# Autodesk Inventor assembly: Track Frame Assembly
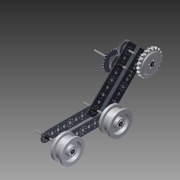
[picture p0: Inventor's stored thumbnail of the model, 180x180]
Saved by Autodesk Inventor 2015 (Build 190159000, 159)
## iProperties
Created: 2015-09-27
Part Number: Track Frame Assembly
Document SubType Name: Assembly
Designer: Jing-Chen
Author: Jing-Chen
## Documents named in this file (14)
- C:\Users\Jing-Chen\Desktop\Bionic Hybrids 2016\Bionic-Hybrids\CAD\Drivetrain\Sub-Assemblies\Track Frame Assembly.iam
- C:\Users\Jing-Chen\Desktop\Bionic Hybrids 2016\Bionic-Hybrids\Stock\Bracket-U9 - 739067.ipt
- C:\Users\Jing-Chen\Desktop\Bionic Hybrids 2016\Bionic-Hybrids\CAD\Drivetrain\Sub-Assemblies\Track Idler Assembly.iam
- C:\Users\Jing-Chen\Desktop\Bionic Hybrids 2016\Bionic-Hybrids\Stock\Axle-100mm - 739088.ipt
- C:\Users\Jing-Chen\Desktop\Bionic Hybrids 2016\Bionic-Hybrids\Stock\Bearing-Thrust - 739091.ipt
- C:\Users\Jing-Chen\Desktop\Bionic Hybrids 2016\Bionic-Hybrids\Stock\Shaft Collar-Setscrew, Axle - 739092.iam
- C:\Users\Jing-Chen\Desktop\Bionic Hybrids 2016\Bionic-Hybrids\Stock\Track Sprocket - 736468.ipt
- C:\Users\Jing-Chen\Desktop\Bionic Hybrids 2016\Bionic-Hybrids\Stock\Shaft Collar-Setscrew, Axle, Mountable - 739172.iam
- C:\Users\Jing-Chen\Desktop\Bionic Hybrids 2016\Bionic-Hybrids\Stock\Plate-9x1 - 739272.ipt
- C:\Users\Jing-Chen\Desktop\Bionic Hybrids 2016\Bionic-Hybrids\Stock\Spacer 3.125mm- 739100.ipt
- C:\Users\Jing-Chen\Desktop\Bionic Hybrids 2016\Bionic-Hybrids\Stock\Gear-40 tooth - 731901.ipt
- C:\Users\Jing-Chen\Desktop\Bionic Hybrids 2016\Bionic-Hybrids\Stock\Plate-1x1 - 739387.ipt
- C:\Users\Jing-Chen\Desktop\Bionic Hybrids 2016\Bionic-Hybrids\Stock\Chain Sprocket-24 tooth - 739169.ipt
- C:\Users\Jing-Chen\Desktop\Bionic Hybrids 2016\Bionic-Hybrids\Stock\Screw 0.5in - 739097.ipt
## Components (36 placed, 13 different names)
1. Bracket-U9 - 739067:1 — Mate:16, Mate:17, Mate:18, Mate:19, Mate:20, Mate:21, Mate:44, Mate:46, Mate:60, Mate:61, Mate:63, Flush:6, Mate:66, Mate:67, Mate:88, Mate:89, Mate:90, Mate:91, Mate:93, Mate:94, Mate:95
2. Track Idler Assembly:1 [sub-assembly] — Mate:2, Flush:1, Mate:43
3. Axle-100mm - 739088:1 — Mate:2, Flush:1, Mate:11, Mate:41
4. Shaft Collar-Setscrew, Axle - 739092:1 [sub-assembly] — Mate:11, Mate:42
5. Track Sprocket - 736468:1 — Mate:13, Mate:15, Mate:23, Mate:24, Mate:105
6. Shaft Collar-Setscrew, Axle, Mountable - 739172:1 [sub-assembly] — Mate:13, Mate:15, Mate:22, Mate:105, Mate:106, Angle:3
7. Plate-9x1 - 739272:1 — Mate:16, Mate:19, Mate:21, Mate:37, Mate:38, Mate:45, Flush:4, Flush:5, Mate:53
8. Plate-9x1 - 739272:2 — Mate:17, Mate:18, Mate:20, Mate:39, Mate:40, Mate:47
9. Axle-100mm - 739088:2 — Mate:22, Flush:2, Mate:58, Mate:92, Mate:99, Mate:100, Mate:101, Angle:2, Angle:3
10. Bearing-Thrust - 739091:4 — Mate:23, Mate:24, Flush:2
11. Bearing-Thrust - 739091:5 — Mate:44, Mate:45, Mate:48, Mate:50
12. Bearing-Thrust - 739091:6 — Mate:39, Mate:40, Mate:41, Mate:42
13. Bearing-Thrust - 739091:10 — Mate:46, Mate:47, Mate:52
14. Bearing-Thrust - 739091:11 — Mate:37, Mate:38, Mate:43
15. Axle-100mm - 739088:3 — Mate:48, Mate:49, Flush:3, Mate:51
16. Track Idler Assembly:2 [sub-assembly] — Mate:49, Mate:50, Flush:3
17. Shaft Collar-Setscrew, Axle - 739092:2 [sub-assembly] — Mate:51, Mate:52
18. Gear-40 tooth - 731901:1 — Mate:55, Mate:57, Mate:64, Rotation:1, Mate:84, Mate:85, Mate:86, Mate:87
19. Gear-40 tooth - 731901:2 — Mate:73, Mate:74, Mate:75, Mate:76, Rotation:1
20. Shaft Collar-Setscrew, Axle, Mountable - 739172:2 [sub-assembly] — Mate:55, Mate:57, Mate:58, Mate:63, Mate:64, Angle:2
21. Shaft Collar-Setscrew, Axle, Mountable - 739172:4 [sub-assembly] — Mate:60, Mate:61, Mate:65, Mate:66, Angle:1
22. Axle-100mm - 739088:4 — Mate:65, Flush:6, Mate:68, Mate:69, Mate:71, Mate:77, Mate:78, Angle:1, Mate:82
23. Plate-1x1 - 739387:1 — Mate:67, Mate:68, Mate:70
24. Bearing-Thrust - 739091:12 — Mate:69, Mate:70, Mate:72
25. Spacer 3.125mm- 739100:3 — Mate:71, Mate:72, Mate:76
26. Shaft Collar-Setscrew, Axle, Mountable - 739172:6 [sub-assembly] — Mate:73, Mate:74, Mate:75, Mate:77, Mate:79, Mate:80, Mate:81
27. Chain Sprocket-24 tooth - 739169:1 — Mate:78, Mate:79, Mate:80, Mate:81, Mate:83
28. Spacer 3.125mm- 739100:4 — Mate:82, Mate:83
29. Screw 0.5in - 739097:1 — Mate:84, Mate:86
30. Screw 0.5in - 739097:2 — Mate:85, Mate:87
31. Screw 0.5in - 739097:3 — Mate:88, Mate:90
32. Screw 0.5in - 739097:4 — Mate:89, Mate:91
33. Shaft Collar-Setscrew, Axle, Mountable - 739172:7 [sub-assembly] — Mate:92, Mate:93, Mate:94, Mate:95, Mate:104
34. Spacer 3.125mm- 739100:5 — Mate:101, Mate:102, Mate:104
35. Spacer 3.125mm- 739100:6 — Mate:100, Mate:102, Mate:103
36. Spacer 3.125mm- 739100:7 — Mate:99, Mate:103, Mate:106
## Relationships (86: Mate 76, Flush 6, Angle 3, RelateRotation 1)
- Mate:2: Track Idler Assembly:1 ↔ Axle-100mm - 739088:1
- Flush:1: Track Idler Assembly:1 ↔ Axle-100mm - 739088:1
- Mate:11: Axle-100mm - 739088:1 ↔ Shaft Collar-Setscrew, Axle - 739092:1
- Mate:13: Track Sprocket - 736468:1 ↔ Shaft Collar-Setscrew, Axle, Mountable - 739172:1
- Mate:15: Track Sprocket - 736468:1 ↔ Shaft Collar-Setscrew, Axle, Mountable - 739172:1
- Mate:16: Bracket-U9 - 739067:1 ↔ Plate-9x1 - 739272:1
- Mate:17: Bracket-U9 - 739067:1 ↔ Plate-9x1 - 739272:2
- Mate:18: Bracket-U9 - 739067:1 ↔ Plate-9x1 - 739272:2
- Mate:19: Bracket-U9 - 739067:1 ↔ Plate-9x1 - 739272:1
- Mate:20: Bracket-U9 - 739067:1 ↔ Plate-9x1 - 739272:2
- Mate:21: Bracket-U9 - 739067:1 ↔ Plate-9x1 - 739272:1
- Mate:22: Shaft Collar-Setscrew, Axle, Mountable - 739172:1 ↔ Axle-100mm - 739088:2
- Mate:23: Track Sprocket - 736468:1 ↔ Bearing-Thrust - 739091:4
- Mate:24: Track Sprocket - 736468:1 ↔ Bearing-Thrust - 739091:4
- Flush:2: Axle-100mm - 739088:2 ↔ Bearing-Thrust - 739091:4
- Mate:37: Plate-9x1 - 739272:1 ↔ Bearing-Thrust - 739091:11
- Mate:38: Plate-9x1 - 739272:1 ↔ Bearing-Thrust - 739091:11
- Mate:39: Plate-9x1 - 739272:2 ↔ Bearing-Thrust - 739091:6
- Mate:40: Plate-9x1 - 739272:2 ↔ Bearing-Thrust - 739091:6
- Mate:41: Axle-100mm - 739088:1 ↔ Bearing-Thrust - 739091:6
- Mate:42: Shaft Collar-Setscrew, Axle - 739092:1 ↔ Bearing-Thrust - 739091:6
- Mate:43: Track Idler Assembly:1 ↔ Bearing-Thrust - 739091:11
- Mate:44: Bracket-U9 - 739067:1 ↔ Bearing-Thrust - 739091:5
- Mate:45: Plate-9x1 - 739272:1 ↔ Bearing-Thrust - 739091:5
- Mate:46: Bracket-U9 - 739067:1 ↔ Bearing-Thrust - 739091:10
- Mate:47: Plate-9x1 - 739272:2 ↔ Bearing-Thrust - 739091:10
- Mate:48: Bearing-Thrust - 739091:5 ↔ Axle-100mm - 739088:3
- Mate:49: Axle-100mm - 739088:3 ↔ Track Idler Assembly:2
- Mate:50: Bearing-Thrust - 739091:5 ↔ Track Idler Assembly:2
- Flush:3: Axle-100mm - 739088:3 ↔ Track Idler Assembly:2
- Mate:51: Axle-100mm - 739088:3 ↔ Shaft Collar-Setscrew, Axle - 739092:2
- Mate:52: Bearing-Thrust - 739091:10 ↔ Shaft Collar-Setscrew, Axle - 739092:2
- Flush:4: Plate-9x1 - 739272:1
- Flush:5: Plate-9x1 - 739272:1
- Mate:53: Plate-9x1 - 739272:1
- Mate:55: Gear-40 tooth - 731901:1 ↔ Shaft Collar-Setscrew, Axle, Mountable - 739172:2
- Mate:57: Gear-40 tooth - 731901:1 ↔ Shaft Collar-Setscrew, Axle, Mountable - 739172:2
- Mate:58: Axle-100mm - 739088:2 ↔ Shaft Collar-Setscrew, Axle, Mountable - 739172:2
- Mate:60: Bracket-U9 - 739067:1 ↔ Shaft Collar-Setscrew, Axle, Mountable - 739172:4
- Mate:61: Bracket-U9 - 739067:1 ↔ Shaft Collar-Setscrew, Axle, Mountable - 739172:4
- Mate:63: Bracket-U9 - 739067:1 ↔ Shaft Collar-Setscrew, Axle, Mountable - 739172:2
- Mate:64: Gear-40 tooth - 731901:1 ↔ Shaft Collar-Setscrew, Axle, Mountable - 739172:2
- Mate:65: Shaft Collar-Setscrew, Axle, Mountable - 739172:4 ↔ Axle-100mm - 739088:4
- Flush:6: Bracket-U9 - 739067:1 ↔ Axle-100mm - 739088:4
- Mate:66: Bracket-U9 - 739067:1 ↔ Shaft Collar-Setscrew, Axle, Mountable - 739172:4
- Mate:67: Bracket-U9 - 739067:1 ↔ Plate-1x1 - 739387:1
- Mate:68: Axle-100mm - 739088:4 ↔ Plate-1x1 - 739387:1
- Mate:69: Axle-100mm - 739088:4 ↔ Bearing-Thrust - 739091:12
- Mate:70: Plate-1x1 - 739387:1 ↔ Bearing-Thrust - 739091:12
- Mate:71: Axle-100mm - 739088:4 ↔ Spacer 3.125mm- 739100:3
- Mate:72: Bearing-Thrust - 739091:12 ↔ Spacer 3.125mm- 739100:3
- Mate:73: Gear-40 tooth - 731901:2 ↔ Shaft Collar-Setscrew, Axle, Mountable - 739172:6
- Mate:74: Gear-40 tooth - 731901:2 ↔ Shaft Collar-Setscrew, Axle, Mountable - 739172:6
- Mate:75: Gear-40 tooth - 731901:2 ↔ Shaft Collar-Setscrew, Axle, Mountable - 739172:6
- Mate:76: Gear-40 tooth - 731901:2 ↔ Spacer 3.125mm- 739100:3
- Mate:77: Axle-100mm - 739088:4 ↔ Shaft Collar-Setscrew, Axle, Mountable - 739172:6
- Rotation:1 [RelateRotation] (1 ul): Gear-40 tooth - 731901:1 ↔ Gear-40 tooth - 731901:2
- Mate:78: Axle-100mm - 739088:4 ↔ Chain Sprocket-24 tooth - 739169:1
- Mate:79: Shaft Collar-Setscrew, Axle, Mountable - 739172:6 ↔ Chain Sprocket-24 tooth - 739169:1
- Mate:80: Shaft Collar-Setscrew, Axle, Mountable - 739172:6 ↔ Chain Sprocket-24 tooth - 739169:1
- Mate:81: Shaft Collar-Setscrew, Axle, Mountable - 739172:6 ↔ Chain Sprocket-24 tooth - 739169:1
- Angle:1 (180 deg): Shaft Collar-Setscrew, Axle, Mountable - 739172:4 ↔ Axle-100mm - 739088:4
- Mate:82: Axle-100mm - 739088:4 ↔ Spacer 3.125mm- 739100:4
- Mate:83: Chain Sprocket-24 tooth - 739169:1 ↔ Spacer 3.125mm- 739100:4
- Mate:84: Gear-40 tooth - 731901:1 ↔ Screw 0.5in - 739097:1
- Mate:85: Gear-40 tooth - 731901:1 ↔ Screw 0.5in - 739097:2
- Mate:86: Gear-40 tooth - 731901:1 ↔ Screw 0.5in - 739097:1
- Mate:87: Gear-40 tooth - 731901:1 ↔ Screw 0.5in - 739097:2
- Mate:88: Bracket-U9 - 739067:1 ↔ Screw 0.5in - 739097:3
- Mate:89: Bracket-U9 - 739067:1 ↔ Screw 0.5in - 739097:4
- Mate:90: Bracket-U9 - 739067:1 ↔ Screw 0.5in - 739097:3
- Mate:91: Bracket-U9 - 739067:1 ↔ Screw 0.5in - 739097:4
- Mate:92: Axle-100mm - 739088:2 ↔ Shaft Collar-Setscrew, Axle, Mountable - 739172:7
- Mate:93: Bracket-U9 - 739067:1 ↔ Shaft Collar-Setscrew, Axle, Mountable - 739172:7
- Mate:94: Bracket-U9 - 739067:1 ↔ Shaft Collar-Setscrew, Axle, Mountable - 739172:7
- Mate:95: Bracket-U9 - 739067:1 ↔ Shaft Collar-Setscrew, Axle, Mountable - 739172:7
- Mate:99: Axle-100mm - 739088:2 ↔ Spacer 3.125mm- 739100:7
- Mate:100: Axle-100mm - 739088:2 ↔ Spacer 3.125mm- 739100:6
- Mate:101: Axle-100mm - 739088:2 ↔ Spacer 3.125mm- 739100:5
- Mate:102: Spacer 3.125mm- 739100:5 ↔ Spacer 3.125mm- 739100:6
- Mate:103: Spacer 3.125mm- 739100:6 ↔ Spacer 3.125mm- 739100:7
- Mate:104: Shaft Collar-Setscrew, Axle, Mountable - 739172:7 ↔ Spacer 3.125mm- 739100:5
- Mate:105: Track Sprocket - 736468:1 ↔ Shaft Collar-Setscrew, Axle, Mountable - 739172:1
- Mate:106: Shaft Collar-Setscrew, Axle, Mountable - 739172:1 ↔ Spacer 3.125mm- 739100:7
- Angle:2 (180 deg): Axle-100mm - 739088:2 ↔ Shaft Collar-Setscrew, Axle, Mountable - 739172:2
- Angle:3 (180 deg): Shaft Collar-Setscrew, Axle, Mountable - 739172:1 ↔ Axle-100mm - 739088:2
